# Autodesk Inventor assembly: caseDoor_rubberSeal
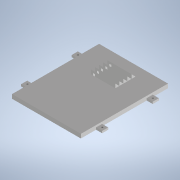
[picture p0: Inventor's stored thumbnail of the model, 180x180]
Saved by Autodesk Inventor 2022.6 (Build 266554010, 554A)
## iProperties
Created: 2025-03-20
Part Number: caseDoor_rubberSeal
Document SubType Name: Assembly
Designer: khinm
Author: khinm
## Documents named in this file (3)
- C:\Users\khinm\Downloads\CAD\toolkit_controllerCaseDesign\caseDoor_rubberSeal.iam
- C:\Users\khinm\Downloads\CAD\caseDoor.ipt
- C:\Users\khinm\Downloads\CAD\rubberSeal.ipt
## Components (2 placed, 2 different names)
1. caseDoor:1 — Mate:1, Mate:2, Mate:3
2. rubberSeal:1 — Mate:1, Mate:2, Mate:3
## Relationships (3: Mate 3)
- Mate:1: caseDoor:1 ↔ rubberSeal:1
- Mate:2: caseDoor:1 ↔ rubberSeal:1
- Mate:3: caseDoor:1 ↔ rubberSeal:1
